# Autodesk Inventor assembly: Motor with Screw Generator
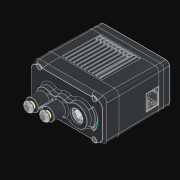
[picture p0: Inventor's stored thumbnail of the model, 180x180]
Saved by Autodesk Inventor 2021.3 (Build 253353010, 353A)
## iProperties
Created: 2021-07-20
Part Number: Motor with Screw Generator
Document SubType Name: Assembly
Designer: yuany
Author: yuany
## Documents named in this file (4)
- E:\VEX Cad\Inventor Library\Electronics\Motors with Screws\Motor with Screw Generator.iam
- E:\VEX Cad\Inventor Library\Electronics\V5 Motor.ipt
- E:\VEX Cad\Inventor Library\Structure\Hardware\Screw Steel - Hex\Screw 8-32 Steel .500.ipt
- E:\VEX Cad\Inventor Library\Structure\Hardware\Screw Steel - Hex.ipt
## Components (3 placed, 2 different names)
1. V5 Motor:1 — Insert:1, Insert:2
2. Screw 8-32 Steel .500:1 — Insert:1
3. Screw 8-32 Steel .500:2 — Insert:2
## Relationships (2: Insert 2)
- Insert:1 (1.6002 mm): V5 Motor:1 ↔ Screw 8-32 Steel .500:1
- Insert:2 (1.6002 mm): V5 Motor:1 ↔ Screw 8-32 Steel .500:2
